# Autodesk Inventor assembly: Assembly2
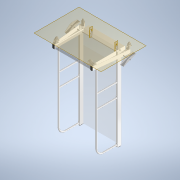
[picture p0: Inventor's stored thumbnail of the model, 180x180]
Saved by Autodesk Inventor 2021 (Build 250183000, 183)
## iProperties
Created: 2026-05-12
Part Number: Assembly2
Document SubType Name: Assembly
Designer: nelso
Author: nelso
## Documents named in this file (8)
- C:\Users\nelso\Desktop\Soporte paciente espinografia\Soporte Paciente Espinografia\Workspaces\Workspace\Assembly2.iam
- C:\Users\nelso\Desktop\Soporte paciente espinografia\Soporte Paciente Espinografia\Workspaces\Workspace\baseChapa.ipt
- C:\Users\nelso\Desktop\Soporte paciente espinografia\Soporte Paciente Espinografia\Workspaces\Workspace\acrilico.ipt
- C:\Users\nelso\Desktop\Soporte paciente espinografia\Soporte Paciente Espinografia\Workspaces\Workspace\Base Ensamblada.iam
- C:\Users\nelso\Desktop\Soporte paciente espinografia\Soporte Paciente Espinografia\Workspaces\Workspace\Baranda Ensamblada.iam
- C:\Users\nelso\Desktop\Soporte paciente espinografia\Soporte Paciente Espinografia\Workspaces\Workspace\DIN933M8X1.25L20C.ipt
- C:\Users\nelso\Desktop\Soporte paciente espinografia\Soporte Paciente Espinografia\Workspaces\Workspace\DIN125-A8,4C.ipt
- C:\Users\nelso\Desktop\Soporte paciente espinografia\Soporte Paciente Espinografia\Workspaces\Workspace\Logo.ipt
## Components (38 placed, 7 different names)
1. baseChapa:1 — Mate:65, Flush:17, Mate:178
2. acrilico:1 — Mate:70, Mate:71, Flush:2
3. Base Ensamblada:1 [sub-assembly] — Flush:1, Mate:71, Flush:2, Coincidencia:97, Coincidencia:98, Coincidencia:99, Coincidencia:100, Coincidencia:101, Coincidencia:102, Coincidencia:117, Nivelación:14, Nivelación:15, Flush:17, Mate:178, Flush:18
4. Baranda Ensamblada:2 [sub-assembly] — Coincidencia:100, Coincidencia:101, Coincidencia:102, Coincidencia:109, Coincidencia:110, Coincidencia:111, Coincidencia:112, Mate:134, Mate:135, Mate:136, Mate:137, Mate:138, Mate:139, Mate:140, Mate:141, Mate:142, Mate:143, Mate:144, Mate:145, Mate:168, Mate:169, Mate:170, Mate:171, Mate:172, Mate:173
5. Baranda Ensamblada:3 [sub-assembly] — Coincidencia:97, Coincidencia:98, Coincidencia:99, Mate:118, Mate:119, Mate:120, Mate:121, Mate:122, Mate:123, Mate:124, Mate:125, Mate:126, Mate:127, Mate:128, Mate:129, Mate:130, Mate:131, Mate:132, Mate:133, Mate:147, Mate:149, Mate:156, Mate:157, Mate:158, Mate:159, Mate:160, Mate:161
6. DIN933M8X1.25L20C:1 — Coincidencia:113, Coincidencia:114
7. DIN125-A8,4C:1 — Coincidencia:109, Coincidencia:110, Coincidencia:115, Coincidencia:116
8. DIN125-A8,4C:2 — Coincidencia:111, Coincidencia:112, Coincidencia:113, Coincidencia:114
9. DIN933M8X1.25L20C:2 — Coincidencia:115, Coincidencia:116
10. Logo:1 — Coincidencia:117, Nivelación:14, Nivelación:15
11. DIN125-A8,4C:3 — Mate:144, Mate:145, Mate:162
12. DIN125-A8,4C:4 — Mate:142, Mate:143, Mate:163
13. DIN125-A8,4C:5 — Mate:140, Mate:141, Mate:164
14. DIN125-A8,4C:6 — Mate:138, Mate:139, Mate:165
15. DIN125-A8,4C:7 — Mate:135, Mate:136, Mate:167
16. DIN125-A8,4C:8 — Mate:134, Mate:137, Mate:166
17. DIN125-A8,4C:9 — Mate:130, Mate:132, Mate:155
18. DIN125-A8,4C:10 — Mate:131, Mate:133, Mate:154
19. DIN125-A8,4C:11 — Mate:128, Mate:129, Mate:153
20. DIN125-A8,4C:12 — Mate:126, Mate:127, Mate:152
21. DIN125-A8,4C:13 — Mate:122, Mate:123, Mate:150
22. DIN125-A8,4C:14 — Mate:124, Mate:125, Mate:151
23. DIN125-A8,4C:15 — Mate:120, Mate:121, Mate:148
24. DIN125-A8,4C:16 — Mate:118, Mate:119, Mate:146
25. DIN933M8X1.25L20C:3 — Mate:162, Mate:168
26. DIN933M8X1.25L20C:4 — Mate:163, Mate:169
27. DIN933M8X1.25L20C:5 — Mate:164, Mate:170
28. DIN933M8X1.25L20C:6 — Mate:165, Mate:171
29. DIN933M8X1.25L20C:7 — Mate:166, Mate:172
30. DIN933M8X1.25L20C:8 — Mate:167, Mate:173
31. DIN933M8X1.25L20C:9 — Mate:155, Mate:156
32. DIN933M8X1.25L20C:10 — Mate:154, Mate:157
33. DIN933M8X1.25L20C:11 — Mate:153, Mate:159
34. DIN933M8X1.25L20C:12 — Mate:152, Mate:158
35. DIN933M8X1.25L20C:13 — Mate:151, Mate:160
36. DIN933M8X1.25L20C:14 — Mate:150, Mate:161
37. DIN933M8X1.25L20C:15 — Mate:148, Mate:149
38. DIN933M8X1.25L20C:16 — Mate:146, Mate:147
## Relationships (81: Mate 75, Flush 6)
- Mate:65: baseChapa:1
- Flush:1: Base Ensamblada:1
- Mate:70: acrilico:1
- Mate:71: acrilico:1 ↔ Base Ensamblada:1
- Flush:2: acrilico:1 ↔ Base Ensamblada:1
- Coincidencia:97 [Mate]: Base Ensamblada:1 ↔ Baranda Ensamblada:3
- Coincidencia:98 [Mate]: Base Ensamblada:1 ↔ Baranda Ensamblada:3
- Coincidencia:99 [Mate]: Base Ensamblada:1 ↔ Baranda Ensamblada:3
- Coincidencia:100 [Mate]: Base Ensamblada:1 ↔ Baranda Ensamblada:2
- Coincidencia:101 [Mate]: Base Ensamblada:1 ↔ Baranda Ensamblada:2
- Coincidencia:102 [Mate]: Base Ensamblada:1 ↔ Baranda Ensamblada:2
- Coincidencia:109 [Mate]: Baranda Ensamblada:2 ↔ DIN125-A8,4C:1
- Coincidencia:110 [Mate]: Baranda Ensamblada:2 ↔ DIN125-A8,4C:1
- Coincidencia:111 [Mate]: Baranda Ensamblada:2 ↔ DIN125-A8,4C:2
- Coincidencia:112 [Mate]: Baranda Ensamblada:2 ↔ DIN125-A8,4C:2
- Coincidencia:113 [Mate]: DIN933M8X1.25L20C:1 ↔ DIN125-A8,4C:2
- Coincidencia:114 [Mate]: DIN933M8X1.25L20C:1 ↔ DIN125-A8,4C:2
- Coincidencia:115 [Mate]: DIN125-A8,4C:1 ↔ DIN933M8X1.25L20C:2
- Coincidencia:116 [Mate]: DIN125-A8,4C:1 ↔ DIN933M8X1.25L20C:2
- Coincidencia:117 [Mate]: Base Ensamblada:1 ↔ Logo:1
- Nivelación:14 [Flush] (10 mm): Base Ensamblada:1 ↔ Logo:1
- Nivelación:15 [Flush] (400 mm): Base Ensamblada:1 ↔ Logo:1
- Mate:118: Baranda Ensamblada:3 ↔ DIN125-A8,4C:16
- Mate:119: Baranda Ensamblada:3 ↔ DIN125-A8,4C:16
- Mate:120: Baranda Ensamblada:3 ↔ DIN125-A8,4C:15
- Mate:121: Baranda Ensamblada:3 ↔ DIN125-A8,4C:15
- Mate:122: Baranda Ensamblada:3 ↔ DIN125-A8,4C:13
- Mate:123: Baranda Ensamblada:3 ↔ DIN125-A8,4C:13
- Mate:124: Baranda Ensamblada:3 ↔ DIN125-A8,4C:14
- Mate:125: Baranda Ensamblada:3 ↔ DIN125-A8,4C:14
- Mate:126: Baranda Ensamblada:3 ↔ DIN125-A8,4C:12
- Mate:127: Baranda Ensamblada:3 ↔ DIN125-A8,4C:12
- Mate:128: Baranda Ensamblada:3 ↔ DIN125-A8,4C:11
- Mate:129: Baranda Ensamblada:3 ↔ DIN125-A8,4C:11
- Mate:130: Baranda Ensamblada:3 ↔ DIN125-A8,4C:9
- Mate:131: Baranda Ensamblada:3 ↔ DIN125-A8,4C:10
- Mate:132: Baranda Ensamblada:3 ↔ DIN125-A8,4C:9
- Mate:133: Baranda Ensamblada:3 ↔ DIN125-A8,4C:10
- Mate:134: Baranda Ensamblada:2 ↔ DIN125-A8,4C:8
- Mate:135: Baranda Ensamblada:2 ↔ DIN125-A8,4C:7
- Mate:136: Baranda Ensamblada:2 ↔ DIN125-A8,4C:7
- Mate:137: Baranda Ensamblada:2 ↔ DIN125-A8,4C:8
- Mate:138: Baranda Ensamblada:2 ↔ DIN125-A8,4C:6
- Mate:139: Baranda Ensamblada:2 ↔ DIN125-A8,4C:6
- Mate:140: Baranda Ensamblada:2 ↔ DIN125-A8,4C:5
- Mate:141: Baranda Ensamblada:2 ↔ DIN125-A8,4C:5
- Mate:142: Baranda Ensamblada:2 ↔ DIN125-A8,4C:4
- Mate:143: Baranda Ensamblada:2 ↔ DIN125-A8,4C:4
- Mate:144: Baranda Ensamblada:2 ↔ DIN125-A8,4C:3
- Mate:145: Baranda Ensamblada:2 ↔ DIN125-A8,4C:3
- Mate:146: DIN125-A8,4C:16 ↔ DIN933M8X1.25L20C:16
- Mate:147: Baranda Ensamblada:3 ↔ DIN933M8X1.25L20C:16
- Mate:148: DIN125-A8,4C:15 ↔ DIN933M8X1.25L20C:15
- Mate:149: Baranda Ensamblada:3 ↔ DIN933M8X1.25L20C:15
- Mate:150: DIN125-A8,4C:13 ↔ DIN933M8X1.25L20C:14
- Mate:151: DIN125-A8,4C:14 ↔ DIN933M8X1.25L20C:13
- Mate:152: DIN125-A8,4C:12 ↔ DIN933M8X1.25L20C:12
- Mate:153: DIN125-A8,4C:11 ↔ DIN933M8X1.25L20C:11
- Mate:154: DIN125-A8,4C:10 ↔ DIN933M8X1.25L20C:10
- Mate:155: DIN125-A8,4C:9 ↔ DIN933M8X1.25L20C:9
- Mate:156: Baranda Ensamblada:3 ↔ DIN933M8X1.25L20C:9
- Mate:157: Baranda Ensamblada:3 ↔ DIN933M8X1.25L20C:10
- Mate:158: Baranda Ensamblada:3 ↔ DIN933M8X1.25L20C:12
- Mate:159: Baranda Ensamblada:3 ↔ DIN933M8X1.25L20C:11
- Mate:160: Baranda Ensamblada:3 ↔ DIN933M8X1.25L20C:13
- Mate:161: Baranda Ensamblada:3 ↔ DIN933M8X1.25L20C:14
- Mate:162: DIN125-A8,4C:3 ↔ DIN933M8X1.25L20C:3
- Mate:163: DIN125-A8,4C:4 ↔ DIN933M8X1.25L20C:4
- Mate:164: DIN125-A8,4C:5 ↔ DIN933M8X1.25L20C:5
- Mate:165: DIN125-A8,4C:6 ↔ DIN933M8X1.25L20C:6
- Mate:166: DIN125-A8,4C:8 ↔ DIN933M8X1.25L20C:7
- Mate:167: DIN125-A8,4C:7 ↔ DIN933M8X1.25L20C:8
- Mate:168: Baranda Ensamblada:2 ↔ DIN933M8X1.25L20C:3
- Mate:169: Baranda Ensamblada:2 ↔ DIN933M8X1.25L20C:4
- Mate:170: Baranda Ensamblada:2 ↔ DIN933M8X1.25L20C:5
- Mate:171: Baranda Ensamblada:2 ↔ DIN933M8X1.25L20C:6
- Mate:172: Baranda Ensamblada:2 ↔ DIN933M8X1.25L20C:7
- Mate:173: Baranda Ensamblada:2 ↔ DIN933M8X1.25L20C:8
- Flush:17: baseChapa:1 ↔ Base Ensamblada:1
- Mate:178 (5 mm): baseChapa:1 ↔ Base Ensamblada:1
- Flush:18: Base Ensamblada:1
